# Autodesk Inventor assembly: 自由輪
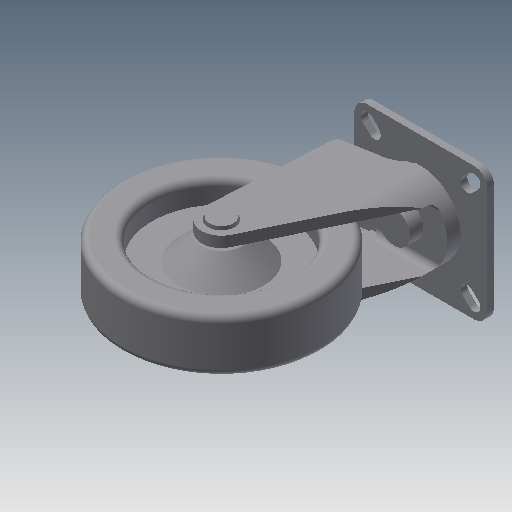
[picture p0: Inventor's stored thumbnail of the model, 512x512]
Saved by Autodesk Inventor 2020.3 (Build 243373000, 373)
## iProperties
Part Number: 自由輪
Material: 一般
Document SubType Name: Assembly
Designer: highs
Description: https://www.monotaro.com/p/3519/5946/
Stock Number: ナンシン プレート式 自在、ゴム(B入り)車 車輪径D 150Φmm、許容荷重 160daN、STC-150CBC
Author: highs
## Documents named in this file (4)
- C:\Users\toshi\Desktop\中の島ex\自由輪.iam
- C:\Users\toshi\Desktop\中の島ex\自由輪パーツ2.ipt
- C:\Users\toshi\Desktop\中の島ex\自由輪パーツ1.ipt
- C:\Users\toshi\Desktop\中の島ex\自由輪パーツ3.ipt
## Components (3 placed, 3 different names)
1. 自由輪パーツ2:1 — メイト:3, メイト:4, 角度:1
2. 自由輪パーツ1:1 — メイト:1, メイト:2, メイト:3, メイト:4, 角度:1
3. 自由輪パーツ3:1 — メイト:1, メイト:2
## Relationships (5: Mate 4, Angle 1)
- メイト:1 [Mate]: 自由輪パーツ1:1 ↔ 自由輪パーツ3:1
- メイト:2 [Mate] (2 mm): 自由輪パーツ1:1 ↔ 自由輪パーツ3:1
- メイト:3 [Mate]: 自由輪パーツ2:1 ↔ 自由輪パーツ1:1
- メイト:4 [Mate]: 自由輪パーツ2:1 ↔ 自由輪パーツ1:1
- 角度:1 [Angle] (0 deg): 自由輪パーツ2:1 ↔ 自由輪パーツ1:1
